# Autodesk Inventor assembly: assembly
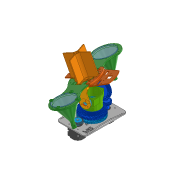
[picture p0: Inventor's stored thumbnail of the model, 180x180]
Saved by Autodesk Inventor 2020.3 (Build 243373000, 373)
## iProperties
Created: 2020-05-02
Part Number: assembly
Description: FreeCAD Model
Document SubType Name: Assembly
Designer: Yusuf
Authority: Unknown
Mass: 501.268 g
Surface Area: 2819.66 cm^2
Volume: 501.268 cm^3
Density: 1 g/cm^3
Sending System: FreeCAD
Preprocessor: Open CASCADE STEP processor 7.3
Title: /home/eyal/data/projects/pan-tilt/mech-design/STEP-files/assembly.step
Author: Author
## Documents named in this file (26)
- C:\Users\Yusuf\Desktop\PanTiltMechanism\assembly.iam
- C:\Users\Yusuf\Desktop\PanTiltMechanism\tilt-arm.ipt
- C:\Users\Yusuf\Desktop\PanTiltMechanism\tilt-pinion.ipt
- C:\Users\Yusuf\Desktop\PanTiltMechanism\pan-pinion.ipt
- C:\Users\Yusuf\Desktop\PanTiltMechanism\base-to-pan-bearings.ipt
- C:\Users\Yusuf\Desktop\PanTiltMechanism\pan-to-tilt-bearings.ipt
- C:\Users\Yusuf\Desktop\PanTiltMechanism\pan-base-gear.ipt
- C:\Users\Yusuf\Desktop\PanTiltMechanism\tilt-base-gear.ipt
- C:\Users\Yusuf\Desktop\PanTiltMechanism\bevel-gear001.ipt
- C:\Users\Yusuf\Desktop\PanTiltMechanism\pan-motor.ipt
- C:\Users\Yusuf\Desktop\PanTiltMechanism\tilt-motor.ipt
- C:\Users\Yusuf\Desktop\PanTiltMechanism\base-plate.ipt
- C:\Users\Yusuf\Desktop\PanTiltMechanism\bevel-gear002.ipt
- C:\Users\Yusuf\Desktop\PanTiltMechanism\turret.ipt
- C:\Users\Yusuf\Desktop\PanTiltMechanism\tilt-arm_MirrorV2.ipt
- C:\Users\Yusuf\Desktop\SunCollector_Autodesk\SunTrackerHolder.ipt
- C:\Users\Yusuf\Desktop\SunCollector_Autodesk\payload-plateV2.ipt
- C:\Users\Yusuf\Desktop\SunCollector_Autodesk\bevel-gear-side.ipt
- C:\Users\Yusuf\Desktop\SunCollector_Autodesk\OneLensHolder.ipt
- C:\Users\Yusuf\Desktop\SunCollector_Autodesk\LensV2.ipt
- C:\Users\Yusuf\Desktop\SunCollector_Autodesk\ClipsForLens.ipt
- C:\Users\Yusuf\Desktop\SunCollector_Autodesk\SensorHolder.ipt
- C:\Users\Yusuf\Desktop\SunCollector_Autodesk\OneLensHolder_MirrorV2.ipt
- C:\Users\Yusuf\Desktop\SunCollector_Autodesk\LensV2_MirrorV2.ipt
- C:\Users\Yusuf\Desktop\SunCollector_Autodesk\ClipsForLens_MirrorV2.ipt
- C:\Users\Yusuf\Desktop\SunCollector_Autodesk\SensorHolderSmall.ipt
## Components (31 placed, 25 different names)
1. tilt-arm — Mate:24, Mate:25, Mate:36, Mate:52, Mate:53
2. tilt-pinion — Flush:3, Mate:35, Rotation:1
3. pan-pinion — Flush:2, Mate:34, Rotation:2
4. base-to-pan-bearings
5. pan-to-tilt-bearings
6. pan-base-gear — Mate:4, Mate:5, Mate:7, Mate:8, Mate:10, Mate:11, Mate:12, Mate:13, Mate:14, Flush:2, Rotation:2
7. tilt-base-gear — Mate:14, Mate:15, Mate:17, Mate:18, Flush:3, Rotation:1, Rotation:3
8. bevel-gear001 — Mate:12, Mate:15, Mate:16, Mate:18
9. pan-motor — Mate:29, Mate:31, Mate:33, Mate:34
10. tilt-motor — Mate:28, Mate:30, Mate:32, Mate:35
11. base-plate — Mate:6, Mate:8, Mate:9, Mate:10, Mate:13, Mate:17, Mate:28, Mate:29, Mate:30, Mate:31, Mate:32, Mate:33
12. bevel-gear002 — Mate:23, Mate:24, Mate:25, Mate:26, Rotation:3, Mate:36
13. turret — Mate:4, Mate:5, Mate:6, Mate:7, Mate:9, Mate:11, Mate:16, Mate:23, Mate:26, Mate:37, Angle:1, Symmetry:1, Mate:55
14. tilt-arm_MirrorV2:1 — Mate:46, Mate:47, Mate:48, Mate:54, Mate:55, Mate:56, Mate:57, Mate:58
15. SunTrackerHolder:1 — Mate:49, Mate:50, Mate:51, Flush:4, Symmetry:2
16. payload-plateV2:1 — Mate:46, Mate:47, Mate:48, Mate:49, Mate:50, Mate:51, Mate:52, Mate:53, Mate:54, Mate:59, Mate:60, Mate:61, Mate:66, Mate:67, Mate:70, Mate:73
17. bevel-gear-side:1 — Mate:56, Mate:57, Mate:58
18. OneLensHolder:1 — Mate:59, Mate:60, Mate:61, Mate:62, Mate:63, Mate:65, Mate:68, Mate:71
19. LensV2:1 — Mate:62, Mate:63, Mate:64
20. SensorHolder:1 — Mate:66, Mate:67, Mate:68, Mate:74
21. OneLensHolder_MirrorV2:1 — Mate:69, Mate:70, Mate:73, Mate:74, Mate:75, Mate:76
22. LensV2_MirrorV2:1 — Mate:69
23. ClipsForLens_MirrorV2:1
24. ClipsForLens_MirrorV2:2
25. ClipsForLens_MirrorV2:3
26. ClipsForLens_MirrorV2:4
27. SensorHolderSmall:1 — Mate:71, Mate:75, Mate:76
28. ClipsForLens:1 — Mate:64, Mate:65
29. ClipsForLens:2
30. ClipsForLens:3
31. ClipsForLens:4
## Component patterns: (4 elements, first: ClipsForLens:1)
## Relationships (68: Mate 59, Flush 3, RelateRotation 3, Symmetry 2, Angle 1)
- Mate:4: pan-base-gear ↔ turret
- Mate:5: pan-base-gear ↔ turret
- Mate:6: base-plate ↔ turret
- Mate:7: pan-base-gear ↔ turret
- Mate:8: pan-base-gear ↔ base-plate
- Mate:9: base-plate ↔ turret
- Mate:10: pan-base-gear ↔ base-plate
- Mate:11: pan-base-gear ↔ turret
- Mate:12: pan-base-gear ↔ bevel-gear001
- Mate:13 (1 mm): pan-base-gear ↔ base-plate
- Mate:14 (1 mm): pan-base-gear ↔ tilt-base-gear
- Mate:15: tilt-base-gear ↔ bevel-gear001
- Mate:16 (0.2 mm): bevel-gear001 ↔ turret
- Mate:17: tilt-base-gear ↔ base-plate
- Mate:18: tilt-base-gear ↔ bevel-gear001
- Mate:23: bevel-gear002 ↔ turret
- Mate:24: tilt-arm ↔ bevel-gear002
- Mate:25: tilt-arm ↔ bevel-gear002
- Mate:26 (1.2 mm): bevel-gear002 ↔ turret
- Mate:28: tilt-motor ↔ base-plate
- Mate:29: pan-motor ↔ base-plate
- Mate:30: tilt-motor ↔ base-plate
- Mate:31: pan-motor ↔ base-plate
- Mate:32: tilt-motor ↔ base-plate
- Mate:33: pan-motor ↔ base-plate
- Flush:2: pan-pinion ↔ pan-base-gear
- Mate:34: pan-pinion ↔ pan-motor
- Flush:3: tilt-pinion ↔ tilt-base-gear
- Mate:35: tilt-pinion ↔ tilt-motor
- Rotation:1 [RelateRotation] (1 ul): tilt-pinion ↔ tilt-base-gear
- Rotation:2 [RelateRotation] (1 ul): pan-pinion ↔ pan-base-gear
- Rotation:3 [RelateRotation] (1 ul): tilt-base-gear ↔ bevel-gear002
- Mate:36: tilt-arm ↔ bevel-gear002
- Mate:37: turret
- Angle:1 (0 deg): turret
- Symmetry:1: turret
- Mate:46: tilt-arm_MirrorV2:1 ↔ payload-plateV2:1
- Mate:47: tilt-arm_MirrorV2:1 ↔ payload-plateV2:1
- Mate:48: tilt-arm_MirrorV2:1 ↔ payload-plateV2:1
- Mate:49: SunTrackerHolder:1 ↔ payload-plateV2:1
- Mate:50: SunTrackerHolder:1 ↔ payload-plateV2:1
- Mate:51: SunTrackerHolder:1 ↔ payload-plateV2:1
- Mate:52: tilt-arm ↔ payload-plateV2:1
- Mate:53: tilt-arm ↔ payload-plateV2:1
- Mate:54: tilt-arm_MirrorV2:1 ↔ payload-plateV2:1
- Mate:55: turret ↔ tilt-arm_MirrorV2:1
- Mate:56: tilt-arm_MirrorV2:1 ↔ bevel-gear-side:1
- Mate:57: tilt-arm_MirrorV2:1 ↔ bevel-gear-side:1
- Mate:58: tilt-arm_MirrorV2:1 ↔ bevel-gear-side:1
- Mate:59: payload-plateV2:1 ↔ OneLensHolder:1
- Mate:60: payload-plateV2:1 ↔ OneLensHolder:1
- Mate:61: payload-plateV2:1 ↔ OneLensHolder:1
- Mate:62: OneLensHolder:1 ↔ LensV2:1
- Mate:63: OneLensHolder:1 ↔ LensV2:1
- Mate:64: LensV2:1 ↔ ClipsForLens:1
- Mate:65: OneLensHolder:1 ↔ ClipsForLens:1
- Mate:66 (4 mm): payload-plateV2:1 ↔ SensorHolder:1
- Mate:67: payload-plateV2:1 ↔ SensorHolder:1
- Mate:68: OneLensHolder:1 ↔ SensorHolder:1
- Flush:4: SunTrackerHolder:1
- Symmetry:2: SunTrackerHolder:1
- Mate:69: OneLensHolder_MirrorV2:1 ↔ LensV2_MirrorV2:1
- Mate:70: payload-plateV2:1 ↔ OneLensHolder_MirrorV2:1
- Mate:71: OneLensHolder:1 ↔ SensorHolderSmall:1
- Mate:73: payload-plateV2:1 ↔ OneLensHolder_MirrorV2:1
- Mate:74: SensorHolder:1 ↔ OneLensHolder_MirrorV2:1
- Mate:75: OneLensHolder_MirrorV2:1 ↔ SensorHolderSmall:1
- Mate:76: OneLensHolder_MirrorV2:1 ↔ SensorHolderSmall:1
